# Autodesk Inventor assembly: xy-mount-assembly(right)1
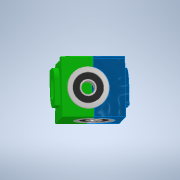
[picture p0: Inventor's stored thumbnail of the model, 180x180]
Saved by Autodesk Inventor 2020.4 (Build 244396000, 396)
## iProperties
Created: 2021-03-01
Part Number: xy-mount-assembly(right)1
Document SubType Name: Assembly
Designer: AOB
Mass: 44.5102 g
Surface Area: 87.5352 cm^2
Volume: 10.3625 cm^3
Density: 4.29533 g/cm^3
Author: AOB
## Documents named in this file (6)
- C:\Users\marti\Documents\Inventor\ProjectBoron\Boron Ultima\xy-mount-assembly(right)1.iam
- xy-mount-assembly(mirror)1.iam
- C:\Users\marti\Documents\Inventor\ProjectBoron\Boron Ultima\xy-mount-bottom(right).ipt
- C:\Users\marti\Documents\Inventor\ProjectBoron\Boron Ultima\xy-mount-top(right)1.ipt
- C:\Users\marti\Documents\Inventor\ProjectBoron\Boron Ultima\688zz bearing.ipt
- C:\Users\marti\Documents\Inventor\ProjectBoron\Boron Ultima\lm8uu-graphite.ipt
## Components (5 placed, 4 different names)
1. xy-mount-bottom(right):1 — Flush:1, Mate:1, Mate:3, Mate:2, Rigid:1
2. 688zz bearing:1 — Flush:2, Mate:6
3. 688zz bearing:2 — Mate:5, Flush:3
4. xy-mount-top(right)1:1 — Flush:1, Mate:1, Mate:4, Flush:2, Mate:5, Flush:3, Mate:6, Rigid:1
5. lm8uu-graphite:1 — Mate:4, Mate:3, Mate:2
## Relationships (10: Mate 6, Flush 3, WeldJoint 1)
- Flush:1: xy-mount-bottom(right):1 ↔ xy-mount-top(right)1:1
- Mate:1: xy-mount-bottom(right):1 ↔ xy-mount-top(right)1:1
- Mate:4: xy-mount-top(right)1:1 ↔ lm8uu-graphite:1
- Mate:3: xy-mount-bottom(right):1 ↔ lm8uu-graphite:1
- Mate:2: xy-mount-bottom(right):1 ↔ lm8uu-graphite:1
- Flush:2: 688zz bearing:1 ↔ xy-mount-top(right)1:1
- Mate:5: 688zz bearing:2 ↔ xy-mount-top(right)1:1
- Flush:3: 688zz bearing:2 ↔ xy-mount-top(right)1:1
- Mate:6: 688zz bearing:1 ↔ xy-mount-top(right)1:1
- Rigid:1 [WeldJoint]: xy-mount-bottom(right):1 ↔ xy-mount-top(right)1:1
